# Autodesk Inventor assembly: BG204_trajan20_21
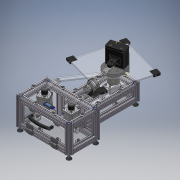
[picture p0: Inventor's stored thumbnail of the model, 180x180]
Saved by Autodesk Inventor 2022.2 (Build 262287000, 287)
## iProperties
Company: HTBLA Kaindorf
RuleStatus: InUse
Created: 2022-09-09
Part Number: BG204_trajan20_21
Project: Zeichenmaschine_v2
Material: Generisch
Description: mit gelenken und stifthalter
Document SubType Name: Assembly
Designer: trajan20
AfterDocNew0: iProperties-Editor_aufrufen
Author: jan
Keywords: 2021
## Documents named in this file (4)
- C:\Users\jan\Documents\DrawMachine\DrawMachineConstruction\Projekt\Zeichenmaschine_v2\BG204_trajan20_21_Zeichenmaschine_v2_mit gelenken und stifthalter.iam
- C:\Users\jan\Documents\DrawMachine\DrawMachineConstruction\Projekt\Zeichenmaschine_v2\BG203_trajan20_21_Zeichenmaschine_v2_Gerüst mit Papierplatte und Seitenwänden.iam
- C:\Users\jan\Documents\DrawMachine\DrawMachineConstruction\Projekt\Zeichenmaschine_v2\BG501_trajan20_21_Zeichenmaschine_v2_Stifthalter.iam
- C:\Users\jan\Documents\DrawMachine\DrawMachineConstruction\Projekt\Zeichenmaschine_v2\BG301_trajan20_21_Zeichenmaschine_v2_gelenke.iam
## Components (3 placed, 3 different names)
1. BG203_trajan20_21_Zeichenmaschine_v2_Gerüst mit Papierplatte und Seitenwänden:1 [sub-assembly] — Passend:1, Passend:2, Passend:3
2. BG501_trajan20_21_Zeichenmaschine_v2_Stifthalter:1 [sub-assembly] — Passend:4, Passend:5, Passend:6
3. BG301_trajan20_21_Zeichenmaschine_v2_gelenke:1 [sub-assembly] — Passend:1, Passend:2, Passend:3, Passend:4, Passend:5, Passend:6
## Relationships (6: Mate 6)
- Passend:1 [Mate]: BG203_trajan20_21_Zeichenmaschine_v2_Gerüst mit Papierplatte und Seitenwänden:1 ↔ BG301_trajan20_21_Zeichenmaschine_v2_gelenke:1
- Passend:2 [Mate]: BG203_trajan20_21_Zeichenmaschine_v2_Gerüst mit Papierplatte und Seitenwänden:1 ↔ BG301_trajan20_21_Zeichenmaschine_v2_gelenke:1
- Passend:3 [Mate]: BG203_trajan20_21_Zeichenmaschine_v2_Gerüst mit Papierplatte und Seitenwänden:1 ↔ BG301_trajan20_21_Zeichenmaschine_v2_gelenke:1
- Passend:4 [Mate]: BG501_trajan20_21_Zeichenmaschine_v2_Stifthalter:1 ↔ BG301_trajan20_21_Zeichenmaschine_v2_gelenke:1
- Passend:5 [Mate]: BG501_trajan20_21_Zeichenmaschine_v2_Stifthalter:1 ↔ BG301_trajan20_21_Zeichenmaschine_v2_gelenke:1
- Passend:6 [Mate]: BG501_trajan20_21_Zeichenmaschine_v2_Stifthalter:1 ↔ BG301_trajan20_21_Zeichenmaschine_v2_gelenke:1
